# Autodesk Inventor assembly: gakutasu-cat-wheel
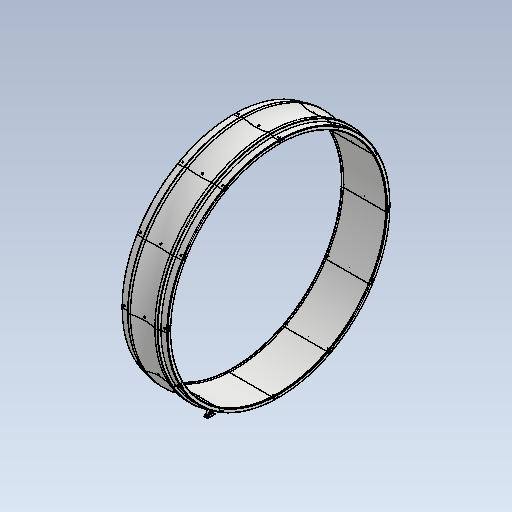
[picture p0: Inventor's stored thumbnail of the model, 512x512]
Saved by Autodesk Inventor 2026.2 (Build 302298010, 298A)
## iProperties
Created: 2026-01-17
Part Number: gakutasu-cat-wheel
Document SubType Name: Assembly
Designer: gakut
Author: gakut
## Documents named in this file (4)
- C:\Users\gakut\Documents\Inventor\gakutasu-cat-wheel\gakutasu-cat-wheel.iam
- C:\Users\gakut\Documents\Inventor\gakutasu-cat-wheel\parts\wheel_plate.ipt
- C:\Users\gakut\Documents\Inventor\gakutasu-cat-wheel\parts\plate_joint_shaft.ipt
- C:\Users\gakut\Documents\Inventor\gakutasu-cat-wheel\parts\caster_d25.ipt
## Components (14 placed, 3 different names)
1. wheel_plate:1 — Mate:1, Flush:1, Mate:2, Mate:3
2. plate_joint_shaft:1 — Mate:1, Flush:1
3. wheel_plate:2 — Mate:2, Mate:3, Mate:6, Mate:7
4. wheel_plate:3 — Mate:6, Mate:7
5. wheel_plate:4 — Mate:14, Mate:15
6. wheel_plate:5 — Mate:14, Mate:15
7. wheel_plate:6
8. wheel_plate:7
9. wheel_plate:8 — Mate:22, Mate:23
10. wheel_plate:9 — Mate:22, Mate:23
11. wheel_plate:10
12. wheel_plate:11
13. wheel_plate:12
14. caster_d25:1
## Relationships (24: Mate 23, Flush 1)
- Mate:1: wheel_plate:1 ↔ plate_joint_shaft:1
- Flush:1: wheel_plate:1 ↔ plate_joint_shaft:1
- Mate:2: wheel_plate:1 ↔ wheel_plate:2
- Mate:3: wheel_plate:1 ↔ wheel_plate:2
- [Mate]: wheel_plate:3 ↔ wheel_plate:4
- [Mate]: wheel_plate:3 ↔ wheel_plate:4
- Mate:6: wheel_plate:2 ↔ wheel_plate:3
- Mate:7: wheel_plate:2 ↔ wheel_plate:3
- [Mate]: wheel_plate:5 ↔ wheel_plate:6
- [Mate]: wheel_plate:5 ↔ wheel_plate:6
- [Mate]: wheel_plate:7 ↔ wheel_plate:8
- [Mate]: wheel_plate:7 ↔ wheel_plate:8
- [Mate]: wheel_plate:6 ↔ wheel_plate:7
- [Mate]: wheel_plate:6 ↔ wheel_plate:7
- Mate:14: wheel_plate:4 ↔ wheel_plate:5
- Mate:15: wheel_plate:4 ↔ wheel_plate:5
- [Mate]: wheel_plate:9 ↔ wheel_plate:10
- [Mate]: wheel_plate:9 ↔ wheel_plate:10
- [Mate]: wheel_plate:11 ↔ wheel_plate:12
- [Mate]: wheel_plate:11 ↔ wheel_plate:12
- [Mate]: wheel_plate:10 ↔ wheel_plate:11
- [Mate]: wheel_plate:10 ↔ wheel_plate:11
- Mate:22: wheel_plate:8 ↔ wheel_plate:9
- Mate:23: wheel_plate:8 ↔ wheel_plate:9
## Named parameters: d32_d30 = 0 mm, d33_d31 = 0 mm, d36_d30 = 0 mm, d37_d31 = 0 mm, d38_d32_d30 = 0 mm, d39_d33_d31 = 0 mm, d40_d34 = 0 mm, d41_d35 = 0 mm, d44_d30 = 0 mm, d45_d31 = 0 mm, d46_d32_d30 = 0 mm, d47_d33_d31 = 0 mm, d48_d34 = 0 mm, d49_d35 = 0 mm
